# Autodesk Inventor assembly: RCT-T004_front_rear_servo_linkage_assembly
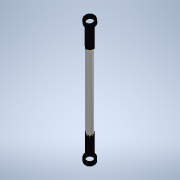
[picture p0: Inventor's stored thumbnail of the model, 180x180]
Saved by Autodesk Inventor 2020 (Build 240168000, 168)
## iProperties
Created: 2019-12-02
Part Number: RCT-T004_front_rear_servo_linkage_assembly
Document SubType Name: Assembly
Designer: maste
Author: maste
## Documents named in this file (3)
- C:\Users\maste\Documents\GitHub\autobot\robot_model\RCT-T004_front_rear_servo_linkage_assembly.iam
- C:\Users\maste\Documents\GitHub\autobot\robot_model\RCT-T004_front_rear_servo_linkage.ipt
- C:\Users\maste\Documents\GitHub\autobot\robot_model\RCT-T003 (2).ipt
## Components (3 placed, 2 different names)
1. RCT-T004_front_rear_servo_linkage:1 — Insert:1, Insert:2
2. RCT-T003 (2):1 — Insert:1
3. RCT-T003 (2):2 — Insert:2
## Relationships (2: Insert 2)
- Insert:1: RCT-T004_front_rear_servo_linkage:1 ↔ RCT-T003 (2):1
- Insert:2: RCT-T004_front_rear_servo_linkage:1 ↔ RCT-T003 (2):2
